# Autodesk Inventor assembly: A1-19037-200-03 34in pipe - flange assy
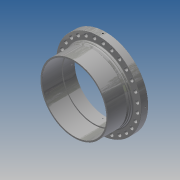
[picture p0: Inventor's stored thumbnail of the model, 180x180]
Saved by Autodesk Inventor 2017.3 (Build 213257000, 257)
## iProperties
Created: 2020-02-10
Part Number: A1-19037-200-03 34in pipe - flange assy
Document SubType Name: Assembly
Designer: KLS
Mass: 421856 g
Surface Area: 34250.5 cm^2
Volume: 53739.7 cm^3
Density: 7.85 g/cm^3
Project: A1-19037--CNUL Albian CST laterals
Constructed By: Krista_Skinner
Project Name: CST laterals
Author: KLS
## Documents named in this file (3)
- C:\156Vault\A1 - Projects\A1-19\A1-19037--CNUL Albian CST laterals\A1-19037-200-03 34in pipe - flange assy.iam
- C:\156Vault\A1 - Projects\A1-19\A1-19037--CNUL Albian CST laterals\A1-19037-200-04 30in CL300 RF flange - custom.ipt
- C:\156Vault\A1 - Projects\A1-19\A1-19037--CNUL Albian CST laterals\A1-19037-200-03 34in pipe.ipt
## Components (2 placed, 2 different names)
1. A1-19037-200-04 30in CL300 RF flange - custom:1
2. A1-19037-200-03 34in pipe:1
## Relationships (2: Insert 1, Angle 1)
- [Insert] (2.3813 mm): A1-19037-200-04 30in CL300 RF flange - custom:1 ↔ A1-19037-200-03 34in pipe:1
- [Angle] (0 deg): A1-19037-200-04 30in CL300 RF flange - custom:1 ↔ A1-19037-200-03 34in pipe:1
